# Autodesk Inventor assembly: Slider
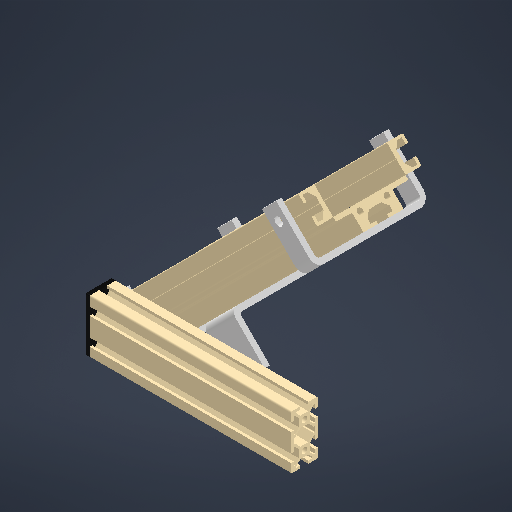
[picture p0: Inventor's stored thumbnail of the model, 512x512]
Saved by Autodesk Inventor 2027 (Build 310192000, 192)
## iProperties
Created: 2026-04-15
Part Number: Slider
Document SubType Name: Assembly
Designer: ratik
Author: ratik
## Documents named in this file (8)
- C:\Users\ratik\OneDrive\Personal Folder\00_Startup\01_Mectosys_Prototype\01_Prototype\01_Mechanical\3D file\Assembly File\Slider.iam
- C:\Users\ratik\OneDrive\Personal Folder\00_Startup\01_Mectosys_Prototype\01_Prototype\01_Mechanical\3D file\02_Slider\08_HFSPURE6-1220-2500_STEP_AP214_20260415\HFSPURE6-1220-2500\HFSPURE6-1220-2500.ipt
- C:\Users\ratik\OneDrive\Personal Folder\00_Startup\01_Mectosys_Prototype\01_Prototype\01_Mechanical\3D file\02_Slider\09_HFSFIN6-1554-1000_STEP_AP214_20260415\HFSFIN6-1554-1000\HFSFIN6-1554-1000.ipt
- C:\Users\ratik\OneDrive\Personal Folder\00_Startup\01_Mectosys_Prototype\01_Prototype\01_Mechanical\3D file\02_Slider\10_HFS5-2040-1500_Inventor\HFS5-2040-1500.ipt
- C:\Users\ratik\OneDrive\Personal Folder\00_Startup\01_Mectosys_Prototype\01_Prototype\01_Mechanical\3D file\02_Slider\08_HFSPURE6-1220-2500_STEP_AP214_20260415\HFSPURE6-1220-2500\HFSPURE6-1220-2500_MIR.ipt
- C:\Users\ratik\OneDrive\Personal Folder\00_Startup\01_Mectosys_Prototype\01_Prototype\01_Mechanical\3D file\02_Slider\11_HFCL5-2040-B_STEP_AP214_20260416\HFCL5-2040-B\HFCL5-2040-B.ipt
- C:\Users\ratik\OneDrive\Personal Folder\00_Startup\01_Mectosys_Prototype\01_Prototype\01_Mechanical\3D file\02_Slider\14_Slider Holding Bracket\Slider Holding Bracket.ipt
- C:\Users\ratik\OneDrive\Personal Folder\00_Startup\01_Mectosys_Prototype\01_Prototype\01_Mechanical\3D file\02_Slider\15_Side bar holding bracket\Side bar holding bracket.ipt
## Components (8 placed, 7 different names)
1. HFS5-2040-1500:1 — Mate:1, Angle:1, Mate:2, Mate:3, Angle:2, Mate:6, Flush:3, Flush:4
2. HFSFIN6-1554-1000:1 — Mate:1, Angle:1, Mate:2, Mate:3, Flush:1, Mate:4, Mate:5, Flush:2, Mate:7, Flush:5, Flush:6, Mate:10
3. HFSPURE6-1220-2500:1 — Angle:2, Flush:1, Mate:11
4. HFSPURE6-1220-2500_MIR:1 — Mate:4, Mate:5, Flush:2, Mate:9, Mate:11, Flush:7
5. HFCL5-2040-B:1 — Mate:6, Flush:3, Flush:4
6. Slider Holding Bracket:1 — Mate:7, Flush:5, Flush:6
7. Side bar holding bracket:1 — Mate:9, Mate:10, Flush:7
8. Side bar holding bracket:2
## Component patterns: (2 elements, first: Side bar holding bracket:1)
## Relationships (19: Mate 10, Flush 7, Angle 2)
- Mate:1 (20 mm): HFS5-2040-1500:1 ↔ HFSFIN6-1554-1000:1
- Angle:1 (45 deg): HFS5-2040-1500:1 ↔ HFSFIN6-1554-1000:1
- Mate:2: HFS5-2040-1500:1 ↔ HFSFIN6-1554-1000:1
- Mate:3: HFS5-2040-1500:1 ↔ HFSFIN6-1554-1000:1
- Angle:2 (45 deg): HFS5-2040-1500:1 ↔ HFSPURE6-1220-2500:1
- Flush:1: HFSFIN6-1554-1000:1 ↔ HFSPURE6-1220-2500:1
- Mate:4: HFSFIN6-1554-1000:1 ↔ HFSPURE6-1220-2500_MIR:1
- Mate:5: HFSFIN6-1554-1000:1 ↔ HFSPURE6-1220-2500_MIR:1
- Flush:2: HFSFIN6-1554-1000:1 ↔ HFSPURE6-1220-2500_MIR:1
- Mate:6: HFS5-2040-1500:1 ↔ HFCL5-2040-B:1
- Flush:3: HFS5-2040-1500:1 ↔ HFCL5-2040-B:1
- Flush:4: HFS5-2040-1500:1 ↔ HFCL5-2040-B:1
- Mate:7: HFSFIN6-1554-1000:1 ↔ Slider Holding Bracket:1
- Flush:5: HFSFIN6-1554-1000:1 ↔ Slider Holding Bracket:1
- Flush:6 (68 mm): HFSFIN6-1554-1000:1 ↔ Slider Holding Bracket:1
- Mate:9: HFSPURE6-1220-2500_MIR:1 ↔ Side bar holding bracket:1
- Mate:10: HFSFIN6-1554-1000:1 ↔ Side bar holding bracket:1
- Mate:11 (54 mm): HFSPURE6-1220-2500:1 ↔ HFSPURE6-1220-2500_MIR:1
- Flush:7 (10 mm): HFSPURE6-1220-2500_MIR:1 ↔ Side bar holding bracket:1
